# Autodesk Inventor assembly: lw_6_сборка
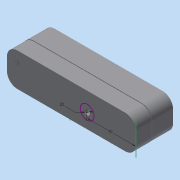
[picture p0: Inventor's stored thumbnail of the model, 180x180]
Saved by Autodesk Inventor 2019 (Build 230136000, 136)
## iProperties
Created: 2021-05-14
Part Number: lw_6_сборка
Material: Типовые
Document SubType Name: Assembly
Designer: Kurbatova
Author: Kurbatova
## Documents named in this file (4)
- C:\Users\Kurbatova\source\LW2021\LW_SAPR\Сборки\lw_6_сборка.iam
- C:\Users\Kurbatova\source\LW2021\LW_SAPR\Детали\lw_6_part1.ipt
- C:\Users\Kurbatova\source\LW2021\LW_SAPR\Детали\lw_6_part2.ipt
- C:\Users\Kurbatova\source\LW2021\LW_SAPR\Сборки\lw_6_сборка\Мастер проектирования\Болтовое соединение1.iam
## Components (3 placed, 3 different names)
1. lw_6_part1:1 — Совмещение:1
2. Болтовое соединение:1 [sub-assembly] — Совмещение:2, Совмещение:3
3. lw_6_part2:1 — Совмещение:1, Совмещение:2, Совмещение:3
## Relationships (3: Mate 3)
- Совмещение:1 [Mate]: lw_6_part1:1 ↔ lw_6_part2:1
- Совмещение:2 [Mate]: Болтовое соединение:1 ↔ lw_6_part2:1
- Совмещение:3 [Mate]: Болтовое соединение:1 ↔ lw_6_part2:1
